# Autodesk Inventor assembly: Fixture_Plate_Assembly
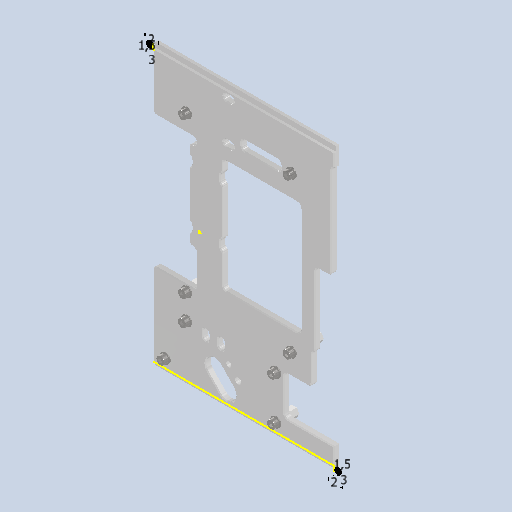
[picture p0: Inventor's stored thumbnail of the model, 512x512]
Saved by Autodesk Inventor 2022 (Build 260153000, 153)
## iProperties
Created: 2020-07-14
Part Number: Fixture_Plate_Assembly
Document SubType Name: Assembly
Designer: CASE-SMALL2
Author: CASE-SMALL2
## Documents named in this file (7)
- C:\Users\Viktor\Documents\GitHub\MARV-Hardware-Mechanical\GPS Base Station\Fixture_Plate\Fixture_Plate_Assembly.iam
- C:\Users\Viktor\Documents\GitHub\MARV-Hardware-Mechanical\GPS Base Station\Fixture_Plate\Fixture_Plate.ipt
- C:\Users\Viktor\Documents\GitHub\MARV-Hardware-Mechanical\GPS Base Station\Fixture_Plate\Standsoffs\M2.5x12mm_Standoff_ 970120144.ipt
- C:\Users\Viktor\Documents\GitHub\MARV-Hardware-Mechanical\GPS Base Station\Fixture_Plate\Standsoffs\M2.5x7mm_Standoff_ 970070151.ipt
- C:\Users\Viktor\Documents\GitHub\MARV-Hardware-Mechanical\GPS Base Station\Fixture_Plate\Screws\DIN 125 - A 2.8.ipt
- C:\Users\Viktor\Documents\GitHub\MARV-Hardware-Mechanical\GPS Base Station\Fixture_Plate\Screws\ISO 4762 - M2.5 x 8ISO.ipt
- C:\Users\Viktor\Documents\GitHub\MARV-Hardware-Mechanical\GPS Base Station\Fixture_Plate\Screws\ISO 4762 - M2.5 x 6ISO.ipt
## Components (25 placed, 6 different names)
1. Fixture_Plate:1 — Rigid:2, Rigid:3, Rigid:5, Rigid:6, Rigid:8, Rigid:9, Rigid:14, Rigid:15, Rigid:16, Rigid:17, Rigid:20, Rigid:31, Rigid:32, Rigid:36, Rigid:34, Rigid:35
2. M2.5x12mm_Standoff_ 970120144:1 — Rigid:35
3. M2.5x12mm_Standoff_ 970120144:2 — Rigid:3
4. M2.5x12mm_Standoff_ 970120144:3 — Rigid:31
5. M2.5x12mm_Standoff_ 970120144:4 — Rigid:2
6. M2.5x7mm_Standoff_ 970070151:1 — Rigid:6
7. M2.5x7mm_Standoff_ 970070151:2 — Rigid:5
8. M2.5x7mm_Standoff_ 970070151:3 — Rigid:9
9. M2.5x7mm_Standoff_ 970070151:4 — Rigid:8
10. DIN 125 - A 2.8:2 — Rigid:29, Rigid:36
11. DIN 125 - A 2.8:3 — Rigid:28, Rigid:32
12. DIN 125 - A 2.8:4 — Rigid:14, Rigid:22
13. DIN 125 - A 2.8:5 — Rigid:15, Rigid:21
14. DIN 125 - A 2.8:6 — Rigid:27, Rigid:34
15. DIN 125 - A 2.8:7 — Rigid:20, Rigid:25
16. DIN 125 - A 2.8:8 — Rigid:17, Rigid:24
17. DIN 125 - A 2.8:10 — Rigid:16, Rigid:23
18. ISO 4762 - M2.5 x 6ISO:1 — Rigid:23
19. ISO 4762 - M2.5 x 6ISO:2 — Rigid:21
20. ISO 4762 - M2.5 x 6ISO:3 — Rigid:24
21. ISO 4762 - M2.5 x 6ISO:4 — Rigid:25
22. ISO 4762 - M2.5 x 8ISO:2 — Rigid:27
23. ISO 4762 - M2.5 x 8ISO:3 — Rigid:22
24. ISO 4762 - M2.5 x 8ISO:4 — Rigid:28
25. ISO 4762 - M2.5 x 8ISO:5 — Rigid:29
## Relationships (24: WeldJoint 24)
- Rigid:2 [WeldJoint]: Fixture_Plate:1 ↔ M2.5x12mm_Standoff_ 970120144:4
- Rigid:3 [WeldJoint]: Fixture_Plate:1 ↔ M2.5x12mm_Standoff_ 970120144:2
- Rigid:5 [WeldJoint]: Fixture_Plate:1 ↔ M2.5x7mm_Standoff_ 970070151:2
- Rigid:6 [WeldJoint]: Fixture_Plate:1 ↔ M2.5x7mm_Standoff_ 970070151:1
- Rigid:8 [WeldJoint]: Fixture_Plate:1 ↔ M2.5x7mm_Standoff_ 970070151:4
- Rigid:9 [WeldJoint]: Fixture_Plate:1 ↔ M2.5x7mm_Standoff_ 970070151:3
- Rigid:14 [WeldJoint]: Fixture_Plate:1 ↔ DIN 125 - A 2.8:4
- Rigid:15 [WeldJoint]: Fixture_Plate:1 ↔ DIN 125 - A 2.8:5
- Rigid:16 [WeldJoint]: Fixture_Plate:1 ↔ DIN 125 - A 2.8:10
- Rigid:17 [WeldJoint]: Fixture_Plate:1 ↔ DIN 125 - A 2.8:8
- Rigid:20 [WeldJoint]: Fixture_Plate:1 ↔ DIN 125 - A 2.8:7
- Rigid:21 [WeldJoint]: DIN 125 - A 2.8:5 ↔ ISO 4762 - M2.5 x 6ISO:2
- Rigid:22 [WeldJoint]: DIN 125 - A 2.8:4 ↔ ISO 4762 - M2.5 x 8ISO:3
- Rigid:23 [WeldJoint]: DIN 125 - A 2.8:10 ↔ ISO 4762 - M2.5 x 6ISO:1
- Rigid:24 [WeldJoint]: DIN 125 - A 2.8:8 ↔ ISO 4762 - M2.5 x 6ISO:3
- Rigid:25 [WeldJoint]: DIN 125 - A 2.8:7 ↔ ISO 4762 - M2.5 x 6ISO:4
- Rigid:27 [WeldJoint]: DIN 125 - A 2.8:6 ↔ ISO 4762 - M2.5 x 8ISO:2
- Rigid:28 [WeldJoint]: DIN 125 - A 2.8:3 ↔ ISO 4762 - M2.5 x 8ISO:4
- Rigid:29 [WeldJoint]: DIN 125 - A 2.8:2 ↔ ISO 4762 - M2.5 x 8ISO:5
- Rigid:31 [WeldJoint]: Fixture_Plate:1 ↔ M2.5x12mm_Standoff_ 970120144:3
- Rigid:32 [WeldJoint]: Fixture_Plate:1 ↔ DIN 125 - A 2.8:3
- Rigid:36 [WeldJoint]: Fixture_Plate:1 ↔ DIN 125 - A 2.8:2
- Rigid:34 [WeldJoint]: Fixture_Plate:1 ↔ DIN 125 - A 2.8:6
- Rigid:35 [WeldJoint]: Fixture_Plate:1 ↔ M2.5x12mm_Standoff_ 970120144:1
